# Autodesk Inventor assembly: M178-PHTM-1000-05-HRDSET
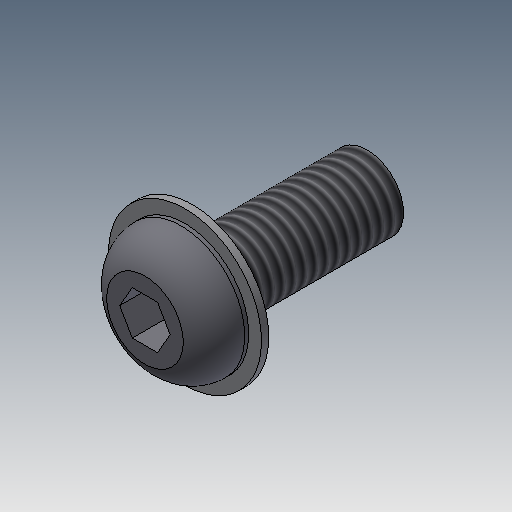
[picture p0: Inventor's stored thumbnail of the model, 512x512]
Saved by Autodesk Inventor 2018.3 (Build 223284000, 284)
## iProperties
Created: 2004-11-19
Part Number: M178-PHTM-1000-05-HRDSET
Document SubType Name: Assembly
Designer: Autodesk, Inc.
Manufacturer: Standard
Standards Organization: Custom
Description: PHANTOM, M10x25 SPRING HARDWARE SET
Mass: 23.1451 g
Surface Area: 21.5811 cm^2
Volume: 3.17882 cm^3
Density: 7.28104 g/cm^3
CAGE: 1LJX3
Dept. ID: Product Design
Description #2: ---
Finish #1: ---
Finish #2: ---
Material ID: ---
Project Number: ---
Author: Autodesk, Inc.
## Documents named in this file (4)
- C:\AVAInvAPI\Workspace\Test Station\Components\M10x25-Spring Phantom.iam
- C:\AVAInvAPI\Workspace\Test Station\Components\24-125-10.ipt
- C:\AVAInvAPI\Workspace\Test Station\Components\24-708-10.ipt
- C:\Users\kelleyb.ADS\Desktop\Samples MIGRATED 2009 224 RTM_1\Standard Parts\Test Station Content\Fastners\2X-YYY-ZZ IPS Screws.ipt
## Components (2 placed, 2 different names)
1. 24-125-10:1
2. 24-708-10:1
## Relationships (1: Insert 1)
- [Insert]: 24-125-10:1 ↔ 24-708-10:1
